# Autodesk Inventor assembly: сборка механизма форточки
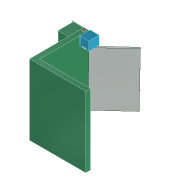
[picture p0: Inventor's stored thumbnail of the model, 180x180]
Saved by Autodesk Inventor 2022 (Build 260153000, 153)
## iProperties
Created: 2023-02-20
Part Number: сборка механизма форточки
Document SubType Name: Assembly
Designer: Egori
Author: Egori
## Documents named in this file (11)
- C:\Теплица\сборка механизма форточки.iam
- C:\Теплица\корпус для серво.ipt
- C:\Теплица\Servo - Tower Pro MG995.ipt
- C:\Теплица\основание форточки.ipt
- C:\Теплица\форточка.ipt
- C:\Теплица\кнопка питания.ipt
- C:\Теплица\WiFi D1 MINI with pins v1.ipt
- C:\Теплица\10pF Ceramic Disc 3.ipt
- C:\Теплица\ACS712.ipt
- C:\Теплица\hlk-pm01.ipt
- C:\Теплица\крышка форточки.ipt
## Components (10 placed, 10 different names)
1. корпус для серво:1 — Совмещение:1, Совмещение:2
2. Servo - Tower Pro MG995:1 — Совмещение:2, С поворотом:1
3. основание форточки:1 — Совмещение:1, Жесткий:1, Совмещение:3, Совмещение:4, Совмещение:5, Совмещение:6, Совмещение:7
4. форточка:1 — С поворотом:1
5. кнопка питания:1 — Жесткий:1
6. WiFi D1 MINI with pins v1:1 — Совмещение:3
7. 10pF Ceramic Disc 3:1 — Совмещение:5
8. ACS712:1 — Совмещение:4
9. hlk-pm01:1 — Совмещение:6
10. крышка форточки:1 — Совмещение:7
## Relationships (9: Mate 7, RevoluteJoint 1, WeldJoint 1)
- Совмещение:1 [Mate]: корпус для серво:1 ↔ основание форточки:1
- Совмещение:2 [Mate]: корпус для серво:1 ↔ Servo - Tower Pro MG995:1
- С поворотом:1 [RevoluteJoint]: Servo - Tower Pro MG995:1 ↔ форточка:1
- Жесткий:1 [WeldJoint]: основание форточки:1 ↔ кнопка питания:1
- Совмещение:3 [Mate]: основание форточки:1 ↔ WiFi D1 MINI with pins v1:1
- Совмещение:4 [Mate]: основание форточки:1 ↔ ACS712:1
- Совмещение:5 [Mate]: основание форточки:1 ↔ 10pF Ceramic Disc 3:1
- Совмещение:6 [Mate]: основание форточки:1 ↔ hlk-pm01:1
- Совмещение:7 [Mate]: основание форточки:1 ↔ крышка форточки:1
